# Autodesk Inventor assembly: FULL SWERVE DRIVE ASSEMBLY!  2!
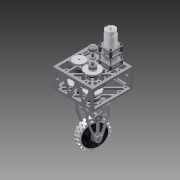
[picture p0: Inventor's stored thumbnail of the model, 180x180]
Saved by Autodesk Inventor 2012 (Build 160160000, 160)
## iProperties
Created: 2013-01-01
Part Number: FULL SWERVE DRIVE ASSEMBLY!  2!
Document SubType Name: Assembly
Designer: Bryce
Author: Bryce
## Documents named in this file (15)
- C:\Users\Bryce\Dropbox\Inventor Design Project Files\Independent Swerves\Inventor 2012\FULL SWERVE DRIVE ASSEMBLY!  2!.iam
- C:\Users\Bryce\Dropbox\Inventor Design Project Files\Independent Swerves\Inventor 2012\upper gearbox frame.ipt
- C:\Users\Bryce\Dropbox\Inventor Design Project Files\Independent Swerves\Inventor 2012\collar bearing systom.ipt
- C:\Users\Bryce\Dropbox\Inventor Design Project Files\Independent Swerves\Inventor 2012\Lower box main assembly 2.iam
- C:\Users\Bryce\Dropbox\Inventor Design Project Files\Independent Swerves\Imported Components\BD Gearbox and Bracket Assy 3.iam
- C:\Users\Bryce\Dropbox\Inventor Design Project Files\Independent Swerves\Imported Components\CIM Motor.iam
- C:\Users\Bryce\Dropbox\Inventor Design Project Files\Independent Swerves\Inventor 2012\turn encoder assembly.iam
- C:\Users\Bryce\Dropbox\Inventor Design Project Files\Independent Swerves\Imported Components\Imported Components\48-5m09-6a5\48-5m09-6a5.ipt
- C:\Users\Bryce\Dropbox\Inventor Design Project Files\Independent Swerves\Inventor 2012\frame assembly 2.iam
- C:\Users\Bryce\Dropbox\Inventor Design Project Files\Independent Swerves\Inventor 2012\frame assembly 3.iam
- C:\Users\Bryce\Dropbox\Inventor Design Project Files\Independent Swerves\Imported Components\0.5'' 15 tooth flange threaded.ipt
- C:\Users\Bryce\Dropbox\Inventor Design Project Files\Independent Swerves\Imported Components\.375 15 tooth flange.ipt
- C:\Users\Bryce\Dropbox\Inventor Design Project Files\Independent Swerves\Imported Components\.375 15 tooth flange short.ipt
- C:\Users\Bryce\Dropbox\Inventor Design Project Files\Independent Swerves\Imported Components\encoder gear drive.ipt
- C:\Users\Bryce\Dropbox\Inventor Design Project Files\Independent Swerves\Imported Components\encoder gear turn.ipt
## Components (16 placed, 14 different names)
1. upper gearbox frame:1 — Mate:1, Mate:2, Mate:3, Mate:4, Mate:6, Mate:11, Mate:15, Mate:16, Mate:17, Mate:18, Mate:20, Mate:21, Mate:22, Angle:2, Mate:24, Mate:25, Mate:26, Mate:27, Flush:5, Flush:6, Mate:40, Mate:41, Angle:4
2. collar bearing systom:1 — Mate:1, Mate:2, Flush:1
3. collar bearing systom:2 — Mate:3, Mate:4, Mate:5
4. Lower box main assembly 2:1 [sub-assembly] — Mate:5, Flush:1, Mate:23, Flush:4, Mate:32, Mate:33, Mate:36, Flush:10, Mate:37, Tangent:1
5. BD Gearbox and Bracket Assy 3:1 [sub-assembly] — Mate:6, Mate:28, Mate:39, Mate:40, Mate:41
6. CIM Motor:1 [sub-assembly] — Mate:11, Mate:20, Mate:21, Mate:22, Mate:29
7. turn encoder assembly:1 [sub-assembly] — Mate:17, Mate:18, Angle:1, Angle:2, Rotation:3, Rotation:4
8. turn encoder assembly:2 [sub-assembly] — Mate:15, Mate:16, Angle:1, Rotation:2
9. encoder gear turn:1 — Mate:36, Flush:10, Rotation:3, Rotation:4
10. 48-5m09-6a5:1 — Mate:23, Flush:4, Flush:7, Rotation:5
11. frame assembly 2:1 [sub-assembly] — Mate:24, Mate:25, Mate:26
12. frame assembly 3:1 [sub-assembly] — Mate:27, Flush:5, Flush:6
13. 0.5'' 15 tooth flange threaded:1 — Mate:28, Flush:7, Mate:39, Rotation:5
14. .375 15 tooth flange:1 — Mate:29, Flush:9, Angle:3
15. encoder gear drive:1 — Mate:37, Mate:38, Rotation:2
16. .375 15 tooth flange short:1 — Mate:32, Mate:33, Flush:9, Angle:3, Mate:38
## Relationships (48: Mate 30, Flush 9, Angle 4, RelateRotation 4, Tangent 1)
- Mate:1: upper gearbox frame:1 ↔ collar bearing systom:1
- Mate:2: upper gearbox frame:1 ↔ collar bearing systom:1
- Mate:3: upper gearbox frame:1 ↔ collar bearing systom:2
- Mate:4: upper gearbox frame:1 ↔ collar bearing systom:2
- Mate:5: collar bearing systom:2 ↔ Lower box main assembly 2:1
- Flush:1 (-1.27 mm): collar bearing systom:1 ↔ Lower box main assembly 2:1
- Mate:6: upper gearbox frame:1 ↔ BD Gearbox and Bracket Assy 3:1
- Mate:11: upper gearbox frame:1 ↔ CIM Motor:1
- Mate:15: upper gearbox frame:1 ↔ turn encoder assembly:2
- Mate:16: upper gearbox frame:1 ↔ turn encoder assembly:2
- Mate:17: upper gearbox frame:1 ↔ turn encoder assembly:1
- Mate:18: upper gearbox frame:1 ↔ turn encoder assembly:1
- [Flush]: turn encoder assembly:1 ↔ encoder gear turn:1
- Mate:20 (3.175 mm): upper gearbox frame:1 ↔ CIM Motor:1
- Mate:21 (9.525 mm): upper gearbox frame:1 ↔ CIM Motor:1
- Mate:22 (9.525 mm): upper gearbox frame:1 ↔ CIM Motor:1
- Mate:23: Lower box main assembly 2:1 ↔ 48-5m09-6a5:1
- Flush:4: Lower box main assembly 2:1 ↔ 48-5m09-6a5:1
- Angle:1 (0 deg): turn encoder assembly:1 ↔ turn encoder assembly:2
- Angle:2 (0 deg): upper gearbox frame:1 ↔ turn encoder assembly:1
- Mate:24: upper gearbox frame:1 ↔ frame assembly 2:1
- Mate:25: upper gearbox frame:1 ↔ frame assembly 2:1
- Mate:26: upper gearbox frame:1 ↔ frame assembly 2:1
- Mate:27: upper gearbox frame:1 ↔ frame assembly 3:1
- Flush:5: upper gearbox frame:1 ↔ frame assembly 3:1
- Flush:6: upper gearbox frame:1 ↔ frame assembly 3:1
- Mate:28: BD Gearbox and Bracket Assy 3:1 ↔ 0.5'' 15 tooth flange threaded:1
- Flush:7: 48-5m09-6a5:1 ↔ 0.5'' 15 tooth flange threaded:1
- Mate:29: CIM Motor:1 ↔ .375 15 tooth flange:1
- [Flush]: turn encoder assembly:2 ↔ encoder gear drive:1
- [Mate]: encoder gear drive:1 ↔ .375 15 tooth flange short:1
- Mate:32: Lower box main assembly 2:1 ↔ .375 15 tooth flange short:1
- Mate:33: Lower box main assembly 2:1 ↔ .375 15 tooth flange short:1
- Flush:9: .375 15 tooth flange:1 ↔ .375 15 tooth flange short:1
- Angle:3 (0 deg): .375 15 tooth flange:1 ↔ .375 15 tooth flange short:1
- Mate:36: Lower box main assembly 2:1 ↔ encoder gear turn:1
- Flush:10: Lower box main assembly 2:1 ↔ encoder gear turn:1
- Mate:37: Lower box main assembly 2:1 ↔ encoder gear drive:1
- Mate:38: encoder gear drive:1 ↔ .375 15 tooth flange short:1
- Rotation:2 [RelateRotation] (1 ul): turn encoder assembly:2 ↔ encoder gear drive:1
- Rotation:3 [RelateRotation] (1 ul): turn encoder assembly:1 ↔ encoder gear turn:1
- Rotation:4 [RelateRotation] (1 ul): turn encoder assembly:1 ↔ encoder gear turn:1
- Mate:39: BD Gearbox and Bracket Assy 3:1 ↔ 0.5'' 15 tooth flange threaded:1
- Mate:40: upper gearbox frame:1 ↔ BD Gearbox and Bracket Assy 3:1
- Mate:41: upper gearbox frame:1 ↔ BD Gearbox and Bracket Assy 3:1
- Rotation:5 [RelateRotation] (0.3333 ul): 48-5m09-6a5:1 ↔ 0.5'' 15 tooth flange threaded:1
- Angle:4 (0 deg): upper gearbox frame:1
- Tangent:1: Lower box main assembly 2:1
